# Autodesk Inventor assembly: Assem1
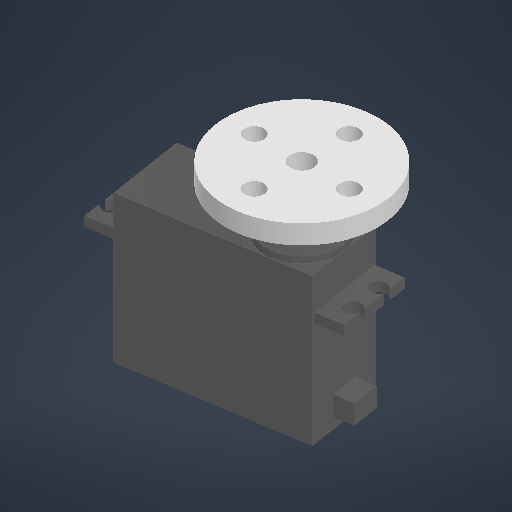
[picture p0: Inventor's stored thumbnail of the model, 512x512]
Saved by Autodesk Inventor 2027.1 (Build 311270010, 270A)
## iProperties
Created: 2021-09-09
Part Number: Assem1
Document SubType Name: Assembly
Designer: daniel
Sending System: SOLIDWORKS 2020
Last Saved Date: 2021-09-09
last saved by: DIMA
Author: daniel
## Documents named in this file (3)
- C:\Ahmed\ASU\Semster 5\DESIGN OF MECHANTRONICS SYSTEMS 1\MCT333_Design_of_Mechatronics_Systems_1\CAD\off_the_shelf_components\standard-servo-motor-black-1.snapshot.7\Assem1\Assem1.iam
- C:\Ahmed\ASU\Semster 5\DESIGN OF MECHANTRONICS SYSTEMS 1\MCT333_Design_of_Mechatronics_Systems_1\CAD\off_the_shelf_components\standard-servo-motor-black-1.snapshot.7\Assem1\body.ipt
- C:\Ahmed\ASU\Semster 5\DESIGN OF MECHANTRONICS SYSTEMS 1\MCT333_Design_of_Mechatronics_Systems_1\CAD\FEED and Sorting\motorShaft Assembly.iam
## Components (2 placed, 2 different names)
1. body-1 — Mate:1, Mate:2
2. motorShaft Assembly:1 [sub-assembly] — Mate:1, Mate:2
## Relationships (2: Mate 2)
- Mate:1: body-1 ↔ motorShaft Assembly:1
- Mate:2: body-1 ↔ motorShaft Assembly:1
